# Autodesk Inventor assembly: shearningMachineAssembly
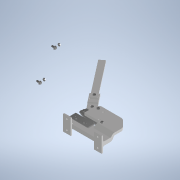
[picture p0: Inventor's stored thumbnail of the model, 180x180]
Saved by Autodesk Inventor 2020.3 (Build 243373000, 373)
## iProperties
Created: 2021-06-19
Part Number: shearningMachineAssembly
Document SubType Name: Assembly
Designer: 0x6f736f646f
Author: 0x6f736f646f
## Documents named in this file (9)
- C:\Users\Public\D\Desktop\Manufacturing-Technology-1-Project\shearningMachineAssembly.iam
- C:\Users\Public\D\Desktop\Manufacturing-Technology-1-Project\body.ipt
- C:\Users\Public\D\Desktop\Manufacturing-Technology-1-Project\Lower blade.ipt
- C:\Users\Public\D\Desktop\Manufacturing-Technology-1-Project\Upper blade.ipt
- C:\Users\Public\D\Desktop\Manufacturing-Technology-1-Project\Support.ipt
- C:\Users\Public\D\Desktop\Manufacturing-Technology-1-Project\handlesupport.ipt
- C:\Users\Public\D\Desktop\Manufacturing-Technology-1-Project\handle.ipt
- C:\Users\Public\D\Desktop\Manufacturing-Technology-1-Project\boltAssembly.iam
- C:\Users\Public\D\Desktop\Manufacturing-Technology-1-Project\Nut.ipt
## Components (24 placed, 8 different names)
1. body:1 — Mate:1, Mate:2, Mate:3, Mate:4, Mate:5, Mate:8, Mate:11, Mate:30, Mate:31, Mate:32, Mate:33, Mate:36, Mate:37, Mate:42, Mate:43
2. Lower blade:1 — Mate:3, Mate:4, Mate:5, Mate:28, Mate:29, Mate:34, Mate:35
3. Upper blade:1 — Mate:1, Mate:2, Mate:6, Mate:7, Mate:27, Mate:38, Mate:40, Mate:41
4. Support:1 — Mate:6, Mate:7, Mate:10, Mate:20, Mate:21, Mate:26
5. handlesupport:1 — Mate:8, Mate:10, Mate:11, Mate:12, Mate:13, Mate:14, Mate:15, Mate:16, Mate:17, Mate:22, Mate:24, Mate:25
6. handle:1 — Mate:12, Mate:13, Mate:14, Mate:15, Mate:19
7. boltAssembly:1 [sub-assembly] — Mate:16, Mate:17, Mate:18
8. Nut:1 — Mate:18, Mate:19
9. boltAssembly:2 [sub-assembly] — Mate:26, Mate:38, Mate:39
10. Nut:2 — Mate:31, Mate:36
11. boltAssembly:3 [sub-assembly] — Mate:24, Mate:25
12. Nut:3 — Mate:30, Mate:37
13. boltAssembly:4 [sub-assembly] — Mate:20, Mate:21, Mate:23
14. Nut:4 — Mate:22, Mate:23
15. boltAssembly:5 [sub-assembly] — Mate:27, Mate:41
16. Nut:5 — Mate:32, Mate:33
17. boltAssembly:6 [sub-assembly]
18. Nut:6
19. boltAssembly:7 [sub-assembly]
20. Nut:7
21. boltAssembly:8 [sub-assembly] — Mate:28, Mate:34
22. Nut:8 — Mate:42, Mate:43
23. boltAssembly:9 [sub-assembly] — Mate:29, Mate:35
24. Nut:9 — Mate:39, Mate:40
## Relationships (42: Mate 42)
- Mate:1: body:1 ↔ Upper blade:1
- Mate:2: body:1 ↔ Upper blade:1
- Mate:3: body:1 ↔ Lower blade:1
- Mate:4: body:1 ↔ Lower blade:1
- Mate:5: body:1 ↔ Lower blade:1
- Mate:6: Upper blade:1 ↔ Support:1
- Mate:7: Upper blade:1 ↔ Support:1
- Mate:8: body:1 ↔ handlesupport:1
- Mate:10: Support:1 ↔ handlesupport:1
- Mate:11: body:1 ↔ handlesupport:1
- Mate:12: handlesupport:1 ↔ handle:1
- Mate:13: handlesupport:1 ↔ handle:1
- Mate:14: handlesupport:1 ↔ handle:1
- Mate:15: handlesupport:1 ↔ handle:1
- Mate:16: handlesupport:1 ↔ boltAssembly:1
- Mate:17: handlesupport:1 ↔ boltAssembly:1
- Mate:18: boltAssembly:1 ↔ Nut:1
- Mate:19: handle:1 ↔ Nut:1
- Mate:20: Support:1 ↔ boltAssembly:4
- Mate:21: Support:1 ↔ boltAssembly:4
- Mate:22: handlesupport:1 ↔ Nut:4
- Mate:23: boltAssembly:4 ↔ Nut:4
- Mate:24: handlesupport:1 ↔ boltAssembly:3
- Mate:25: handlesupport:1 ↔ boltAssembly:3
- Mate:26: Support:1 ↔ boltAssembly:2
- Mate:27: Upper blade:1 ↔ boltAssembly:5
- Mate:28: Lower blade:1 ↔ boltAssembly:8
- Mate:29: Lower blade:1 ↔ boltAssembly:9
- Mate:30: body:1 ↔ Nut:3
- Mate:31: body:1 ↔ Nut:2
- Mate:32: body:1 ↔ Nut:5
- Mate:33: body:1 ↔ Nut:5
- Mate:34: Lower blade:1 ↔ boltAssembly:8
- Mate:35: Lower blade:1 ↔ boltAssembly:9
- Mate:36: body:1 ↔ Nut:2
- Mate:37: body:1 ↔ Nut:3
- Mate:38: Upper blade:1 ↔ boltAssembly:2
- Mate:39: boltAssembly:2 ↔ Nut:9
- Mate:40: Upper blade:1 ↔ Nut:9
- Mate:41: Upper blade:1 ↔ boltAssembly:5
- Mate:42: body:1 ↔ Nut:8
- Mate:43: body:1 ↔ Nut:8
